# Autodesk Inventor assembly: 3drag
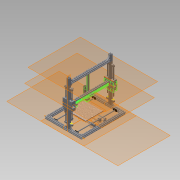
[picture p0: Inventor's stored thumbnail of the model, 180x180]
Saved by Autodesk Inventor 2014 SP1 (Build 180222100, 222)
## iProperties
Created: 2015-04-08
Part Number: 3drag
Document SubType Name: Assembly
Designer: Giorgio Nuzzo
Author: Giorgio Nuzzo
## Documents named in this file (35)
- C:\Users\Giorgio Nuzzo\Desktop\WeMake\total kase\3dragmodel\3drag.iam
- C:\Users\Giorgio Nuzzo\Desktop\WeMake\total kase\3dragmodel\profilato416.ipt
- C:\Users\Giorgio Nuzzo\Desktop\WeMake\total kase\3dragmodel\profilato450.ipt
- C:\Users\Giorgio Nuzzo\Desktop\WeMake\total kase\3dragmodel\angolo-profilati.ipt
- C:\Users\Giorgio Nuzzo\Desktop\WeMake\total kase\3dragmodel\angolo-profilati_MIR.ipt
- C:\Users\Giorgio Nuzzo\Desktop\WeMake\total kase\3dragmodel\angolo-profilati_MIR1.ipt
- C:\Users\Giorgio Nuzzo\Desktop\WeMake\total kase\3dragmodel\angolo-profilati_MIR_MIR.ipt
- C:\Users\Giorgio Nuzzo\Desktop\WeMake\total kase\3dragmodel\profilato500.ipt
- C:\Users\Giorgio Nuzzo\Desktop\WeMake\total kase\3dragmodel\profilato500_MIR1.ipt
- C:\Users\Giorgio Nuzzo\Desktop\WeMake\total kase\3dragmodel\angolo-profilati_MIR3.ipt
- C:\Users\Giorgio Nuzzo\Desktop\WeMake\total kase\3dragmodel\angolo-profilati_MIR4.ipt
- C:\Users\Giorgio Nuzzo\Desktop\WeMake\total kase\3dragmodel\x axys.iam
- C:\Users\Giorgio Nuzzo\Desktop\WeMake\total kase\3dragmodel\Y axys.iam
- C:\Users\Giorgio Nuzzo\Desktop\WeMake\total kase\3dragmodel\z_axys.iam
- C:\Users\Giorgio Nuzzo\Desktop\WeMake\total kase\3dragmodel\z_axys_MIR.iam
- C:\Users\Giorgio Nuzzo\Desktop\WeMake\total kase\3dragmodel\piastra_manicotti.ipt
- C:\Users\Giorgio Nuzzo\Desktop\WeMake\total kase\3dragmodel\supporto_manicotto_Z.ipt
- C:\Users\Giorgio Nuzzo\Desktop\WeMake\total kase\3dragmodel\supporto_manicotto_Z_MIR.ipt
- C:\Users\Giorgio Nuzzo\Desktop\WeMake\total kase\3dragmodel\supporto_manicotto_Z_MIR1.ipt
- C:\Users\Giorgio Nuzzo\Desktop\WeMake\total kase\3dragmodel\supporto_manicotto_Z_MIR_MIR.ipt
- C:\Users\Giorgio Nuzzo\Desktop\WeMake\total kase\3dragmodel\z_axys_MIR1.iam
- C:\Users\Giorgio Nuzzo\Desktop\WeMake\total kase\3dragmodel\z_axys_MIR_MIR.iam
- C:\Users\Giorgio Nuzzo\Desktop\WeMake\total kase\3dragmodel\piastra_manicotti_MIR.ipt
- C:\Users\Giorgio Nuzzo\Desktop\WeMake\total kase\3dragmodel\supporto_manicotto_Z_MIR2.ipt
- C:\Users\Giorgio Nuzzo\Desktop\WeMake\total kase\3dragmodel\supporto_manicotto_Z_MIR_MIR1.ipt
- C:\Users\Giorgio Nuzzo\Desktop\WeMake\total kase\3dragmodel\supporto_manicotto_Z_MIR1_MIR.ipt
- C:\Users\Giorgio Nuzzo\Desktop\WeMake\total kase\3dragmodel\supporto_manicotto_Z_MIR_MIR_MIR.ipt
- C:\Users\Giorgio Nuzzo\Desktop\WeMake\total kase\3dragmodel\z_axys_extrusorù.iam
- C:\Users\Giorgio Nuzzo\Desktop\WeMake\total kase\3dragmodel\angolo-profilati_MIR5.ipt
- C:\Users\Giorgio Nuzzo\Desktop\WeMake\total kase\3dragmodel\giunto_barra_estrusore.ipt
- C:\Users\Giorgio Nuzzo\Desktop\WeMake\total kase\3dragmodel\profilato450estrusore.ipt
- C:\Users\Giorgio Nuzzo\Desktop\WeMake\total kase\3dragmodel\staffa_estrusore.ipt
- C:\Users\Giorgio Nuzzo\Desktop\WeMake\total kase\3dragmodel\profilo_estrusore.ipt
- C:\Users\Giorgio Nuzzo\Desktop\WeMake\total kase\3dragmodel\tubo_coprisiringa.ipt
- C:\Users\Giorgio Nuzzo\Desktop\WeMake\total kase\3dragmodel\giunto_fondo_siringa.ipt
## Components (44 placed, 34 different names)
1. profilato416:1 — Mate:1, Mate:3, Mate:5, Mate:6, Flush:5, Flush:6, Flush:7, Mate:34
2. profilato416:2 — Mate:2, Mate:4, Mate:5, Mate:7, Mate:8, Flush:1, Flush:2, Flush:3, Flush:4
3. profilato450:1 — Mate:8, Flush:1, Flush:4, Mate:12, Mate:13, Mate:16, Flush:10
4. profilato450:2 — Mate:7, Flush:2, Flush:3
5. angolo-profilati:1 — Flush:5
6. angolo-profilati_MIR:1
7. angolo-profilati_MIR1:1
8. angolo-profilati_MIR_MIR:1
9. profilato500:1 — Mate:12, Mate:14, Mate:15, Mate:17, Mate:18, Flush:6, Flush:7, Mate:23, Flush:8, Flush:9, Mate:24, Mate:26, Mate:28, Mate:29, Flush:11
10. angolo-profilati:2 — Mate:13, Mate:14, Mate:15
11. angolo-profilati:3 — Mate:16, Mate:17, Mate:18
12. profilato500_MIR1:1 — Mate:19, Mate:20, Mate:21, Mate:22, Mate:37, Mate:39, Mate:40, Mate:42, Mate:43, Mate:47, Mate:49
13. angolo-profilati_MIR3:1 — Mate:19, Mate:20
14. angolo-profilati_MIR3:2 — Mate:21, Mate:22, Mate:41
15. profilato450:3 — Mate:23, Flush:8, Flush:9, Mate:27, Mate:35, Mate:36
16. angolo-profilati:4 — Mate:27, Mate:28, Mate:29
17. angolo-profilati:5 — Mate:24, Mate:26, Flush:11
18. angolo-profilati_MIR4:2 — Mate:35, Mate:36, Mate:37
19. x axys:1 [sub-assembly] — Mate:32, Mate:33, Mate:34, Angle:2, Insert:1
20. Y axys:1 [sub-assembly] — Angle:2, Insert:1
21. z_axys:1 [sub-assembly] — Mate:39, Mate:40, Mate:41
22. z_axys_MIR:1 [sub-assembly]
23. piastra_manicotti:1 — Mate:42, Mate:43, Mate:44, Flush:12, Flush:13
24. piastra_manicotti:2 — Mate:44, Flush:12, Flush:13, Flush:14
25. supporto_manicotto_Z:1 — Flush:14
26. supporto_manicotto_Z_MIR:1
27. supporto_manicotto_Z_MIR1:1
28. supporto_manicotto_Z_MIR_MIR:1
29. z_axys_MIR1:1 [sub-assembly]
30. z_axys_MIR_MIR:1 [sub-assembly]
31. piastra_manicotti_MIR:1 — Flush:15, Flush:16, Mate:45
32. piastra_manicotti_MIR:2 — Flush:15, Flush:16, Mate:45, Mate:46
33. supporto_manicotto_Z_MIR2:1 — Mate:46
34. supporto_manicotto_Z_MIR_MIR1:1
35. supporto_manicotto_Z_MIR1_MIR:1
36. supporto_manicotto_Z_MIR_MIR_MIR:1
37. z_axys_extrusorù:1 [sub-assembly] — Mate:47, Mate:49, Mate:50, Angle:3
38. angolo-profilati_MIR5:1
39. giunto_barra_estrusore:1 — Mate:50, Angle:3, Mate:51, Mate:52, Mate:53
40. profilato450estrusore:1 — Mate:51, Mate:52, Mate:53, Mate:54, Mate:55, Mate:56
41. staffa_estrusore:1 — Mate:54, Mate:55, Mate:56, Mate:57, Mate:58, Flush:17
42. profilo_estrusore:1 — Mate:57, Mate:58, Flush:17, Flush:18, Mate:59, Mate:60
43. tubo_coprisiringa:1 — Flush:18, Mate:59, Mate:60, Flush:19
44. giunto_fondo_siringa:1 — Flush:19
## Relationships (74: Mate 52, Flush 19, Angle 2, Insert 1)
- Mate:1: profilato416:1
- Mate:2: profilato416:2
- Mate:3: profilato416:1
- Mate:4: profilato416:2
- Mate:5 (450 mm): profilato416:1 ↔ profilato416:2
- Mate:6 (225 mm): profilato416:1
- Mate:7: profilato416:2 ↔ profilato450:2
- Mate:8: profilato416:2 ↔ profilato450:1
- Flush:1: profilato416:2 ↔ profilato450:1
- Flush:2: profilato416:2 ↔ profilato450:2
- Flush:3: profilato416:2 ↔ profilato450:2
- Flush:4: profilato416:2 ↔ profilato450:1
- Flush:5 (-5 mm): profilato416:1 ↔ angolo-profilati:1
- Mate:12: profilato450:1 ↔ profilato500:1
- Mate:13: profilato450:1 ↔ angolo-profilati:2
- Mate:14: profilato500:1 ↔ angolo-profilati:2
- Mate:15: profilato500:1 ↔ angolo-profilati:2
- Mate:16: profilato450:1 ↔ angolo-profilati:3
- Mate:17: profilato500:1 ↔ angolo-profilati:3
- Mate:18: profilato500:1 ↔ angolo-profilati:3
- Flush:6: profilato416:1 ↔ profilato500:1
- Flush:7 (145 mm): profilato416:1 ↔ profilato500:1
- Mate:19: profilato500_MIR1:1 ↔ angolo-profilati_MIR3:1
- Mate:20: profilato500_MIR1:1 ↔ angolo-profilati_MIR3:1
- Mate:21: profilato500_MIR1:1 ↔ angolo-profilati_MIR3:2
- Mate:22: profilato500_MIR1:1 ↔ angolo-profilati_MIR3:2
- Mate:23: profilato500:1 ↔ profilato450:3
- Flush:8: profilato500:1 ↔ profilato450:3
- Flush:9 (40 mm): profilato500:1 ↔ profilato450:3
- Mate:24: profilato500:1 ↔ angolo-profilati:5
- Mate:26: profilato500:1 ↔ angolo-profilati:5
- Mate:27: profilato450:3 ↔ angolo-profilati:4
- Mate:28: profilato500:1 ↔ angolo-profilati:4
- Mate:29: profilato500:1 ↔ angolo-profilati:4
- Flush:10: profilato450:1
- Mate:32: x axys:1
- Mate:33: x axys:1
- Mate:34: profilato416:1 ↔ x axys:1
- Mate:35: profilato450:3 ↔ angolo-profilati_MIR4:2
- Mate:36: profilato450:3 ↔ angolo-profilati_MIR4:2
- Mate:37: profilato500_MIR1:1 ↔ angolo-profilati_MIR4:2
- Flush:11: profilato500:1 ↔ angolo-profilati:5
- Angle:2 (0 deg): x axys:1 ↔ Y axys:1
- Mate:39: profilato500_MIR1:1 ↔ z_axys:1
- Mate:40: profilato500_MIR1:1 ↔ z_axys:1
- Mate:41 (1 mm): angolo-profilati_MIR3:2 ↔ z_axys:1
- Mate:42 (1 mm): profilato500_MIR1:1 ↔ piastra_manicotti:1
- Mate:43: profilato500_MIR1:1 ↔ piastra_manicotti:1
- Mate:44 (38 mm): piastra_manicotti:1 ↔ piastra_manicotti:2
- Flush:12: piastra_manicotti:1 ↔ piastra_manicotti:2
- Flush:13: piastra_manicotti:1 ↔ piastra_manicotti:2
- Flush:14: piastra_manicotti:2 ↔ supporto_manicotto_Z:1
- Flush:15: piastra_manicotti_MIR:1 ↔ piastra_manicotti_MIR:2
- Flush:16: piastra_manicotti_MIR:1 ↔ piastra_manicotti_MIR:2
- Mate:45 (38 mm): piastra_manicotti_MIR:1 ↔ piastra_manicotti_MIR:2
- Mate:46: piastra_manicotti_MIR:2 ↔ supporto_manicotto_Z_MIR2:1
- Insert:1 (-5 mm): x axys:1 ↔ Y axys:1
- Mate:47: profilato500_MIR1:1 ↔ z_axys_extrusorù:1
- Mate:49: profilato500_MIR1:1 ↔ z_axys_extrusorù:1
- Mate:50: z_axys_extrusorù:1 ↔ giunto_barra_estrusore:1
- Angle:3 (0 deg): z_axys_extrusorù:1 ↔ giunto_barra_estrusore:1
- Mate:51: giunto_barra_estrusore:1 ↔ profilato450estrusore:1
- Mate:52: giunto_barra_estrusore:1 ↔ profilato450estrusore:1
- Mate:53: giunto_barra_estrusore:1 ↔ profilato450estrusore:1
- Mate:54: profilato450estrusore:1 ↔ staffa_estrusore:1
- Mate:55: profilato450estrusore:1 ↔ staffa_estrusore:1
- Mate:56 (197.5 mm): profilato450estrusore:1 ↔ staffa_estrusore:1
- Mate:57: staffa_estrusore:1 ↔ profilo_estrusore:1
- Mate:58 (6.5 mm): staffa_estrusore:1 ↔ profilo_estrusore:1
- Flush:17 (-35 mm): staffa_estrusore:1 ↔ profilo_estrusore:1
- Flush:18: profilo_estrusore:1 ↔ tubo_coprisiringa:1
- Mate:59: profilo_estrusore:1 ↔ tubo_coprisiringa:1
- Mate:60 (-30 mm): profilo_estrusore:1 ↔ tubo_coprisiringa:1
- Flush:19 (-2 mm): tubo_coprisiringa:1 ↔ giunto_fondo_siringa:1
